# Autodesk Inventor assembly: AnglePlate
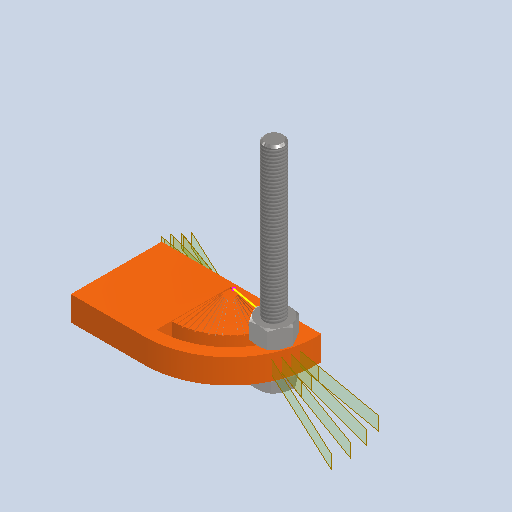
[picture p0: Inventor's stored thumbnail of the model, 512x512]
Saved by Autodesk Inventor 2025.2 (Build 292293000, 293)
## iProperties
Created: 2025-03-13
Part Number: AnglePlate
Document SubType Name: Assembly
Designer: baolo
Author: baolo
## Documents named in this file (4)
- C:\Users\baolo\OneDrive\Desktop\the 2024 homework folder\engg 160\Trebuchet Models\AnglePlate.iam
- C:\Users\baolo\OneDrive\Desktop\the 2024 homework folder\engg 160\Trebuchet Models\MainAnglePlate.ipt
- C:\Users\baolo\OneDrive\Documents\Inventor\Content Center Files\R2025\en-US\BS EN ISO 4017\BS EN ISO 4017 - M8 x 80BS EN.ipt
- C:\Users\baolo\OneDrive\Documents\Inventor\Content Center Files\R2025\en-US\ANSI B 18.2.4.1 M(1)\ANSI B 18.2.4.1 M - M8 x 1.25Style 2.ipt
## Components (3 placed, 3 different names)
1. MainAnglePlate:1 — Flush:1, Mate:2, Flush:2, Mate:5, Angle:1, Angle:2, Angle:3, Angle:4, Mate:10, Tangent:2, Mate:11, Angle:5, Mate:12, Angle:6, Mate:13, Angle:7
2. BS EN ISO 4017 - Metric M8 x 80:1 — Mate:4, Tangent:1, Mate:10, Tangent:2, Tangent:3
3. Hex Nut Metric M8 x 1.25:1 — Mate:4, Mate:5
## Relationships (19: Mate 7, Angle 7, Tangent 3, Flush 2)
- Flush:1: MainAnglePlate:1
- Mate:2: MainAnglePlate:1
- Flush:2: MainAnglePlate:1
- Mate:4: BS EN ISO 4017 - Metric M8 x 80:1 ↔ Hex Nut Metric M8 x 1.25:1
- Mate:5: MainAnglePlate:1 ↔ Hex Nut Metric M8 x 1.25:1
- Angle:1 (0 deg): MainAnglePlate:1
- Angle:2 (0 deg): MainAnglePlate:1
- Angle:3 (0 deg): MainAnglePlate:1
- Angle:4 (0 deg): MainAnglePlate:1
- Tangent:1: BS EN ISO 4017 - Metric M8 x 80:1
- Mate:10: MainAnglePlate:1 ↔ BS EN ISO 4017 - Metric M8 x 80:1
- Tangent:2: MainAnglePlate:1 ↔ BS EN ISO 4017 - Metric M8 x 80:1
- Mate:11: MainAnglePlate:1
- Angle:5 (0 deg): MainAnglePlate:1
- Mate:12: MainAnglePlate:1
- Angle:6 (0 deg): MainAnglePlate:1
- Mate:13: MainAnglePlate:1
- Angle:7 (0 deg): MainAnglePlate:1
- Tangent:3: BS EN ISO 4017 - Metric M8 x 80:1
